# Autodesk Inventor assembly: Hopper Rest 8-32
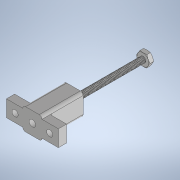
[picture p0: Inventor's stored thumbnail of the model, 180x180]
Saved by Autodesk Inventor 2022.1 (Build 261234020, 234B)
## iProperties
Created: 2021-06-04
Part Number: Hopper Rest 8-32
Document SubType Name: Assembly
Designer: John
Author: John
## Documents named in this file (4)
- C:\Users\muham\Desktop\P3_Complete_Revamp\_Cad models\Autodesk Inventor Files\6. Misc Parts\Resting Block\Hopper Rest 8-32.iam
- C:\Users\muham\Desktop\P3_Complete_Revamp\_Cad models\Autodesk Inventor Files\6. Misc Parts\Resting Block\Hopper Rest Metric Wide.ipt
- C:\Users\muham\Desktop\P3_Complete_Revamp\_Cad models\Autodesk Inventor Files\6. Misc Parts\Resting Block\8-32 x 3 Inch Threaded Rod.ipt
- C:\Users\muham\Desktop\P3_Complete_Revamp\_Cad models\Autodesk Inventor Files\6. Misc Parts\Resting Block\8-32 Hex Nut.ipt
## Components (4 placed, 3 different names)
1. Hopper Rest Metric Wide:1 — Angle:1, Mate:1, Mate:2, Mate:4, Flush:2
2. 8-32 x 3 Inch Threaded Rod:1 — Mate:3, Flush:1, Mate:4, Flush:2
3. 8-32 Hex Nut:1 — Angle:1, Mate:1, Mate:2
4. 8-32 Hex Nut:2 — Mate:3, Flush:1
## Relationships (7: Mate 4, Flush 2, Angle 1)
- Angle:1 (0 deg): Hopper Rest Metric Wide:1 ↔ 8-32 Hex Nut:1
- Mate:1: Hopper Rest Metric Wide:1 ↔ 8-32 Hex Nut:1
- Mate:2: Hopper Rest Metric Wide:1 ↔ 8-32 Hex Nut:1
- Mate:3: 8-32 x 3 Inch Threaded Rod:1 ↔ 8-32 Hex Nut:2
- Flush:1: 8-32 x 3 Inch Threaded Rod:1 ↔ 8-32 Hex Nut:2
- Mate:4: Hopper Rest Metric Wide:1 ↔ 8-32 x 3 Inch Threaded Rod:1
- Flush:2: Hopper Rest Metric Wide:1 ↔ 8-32 x 3 Inch Threaded Rod:1
